# Autodesk Inventor assembly: GFRP_T2_02
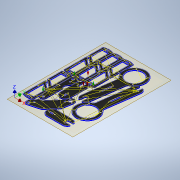
[picture p0: Inventor's stored thumbnail of the model, 180x180]
Saved by Autodesk Inventor 2022 (Build 260153000, 153)
## iProperties
Created: 2022-09-28
Part Number: GFRP_T2_02
Document SubType Name: Assembly
Designer: Masato
Author: Masato
## Documents named in this file (7)
- C:\Users\ヨコオリク\Documents\CITBrains\SUSTAINA-OP\Cam\GFRP_T2\OriginalMind_RD400\GFRP_T2_02.iam
- C:\Users\ヨコオリク\Documents\CITBrains\SUSTAINA-OP\Cam\DisposableBoard.ipt
- C:\Users\ヨコオリク\Documents\CITBrains\SUSTAINA-OP\LowerBody\Link\BackLink_frame.ipt
- C:\Users\ヨコオリク\Documents\CITBrains\SUSTAINA-OP\LowerBody\Link\FrontLink_frame.ipt
- C:\Users\ヨコオリク\Documents\CITBrains\SUSTAINA-OP\UpperBody\Arm\ForeArm_inside_frame.ipt
- C:\Users\ヨコオリク\Documents\CITBrains\SUSTAINA-OP\UpperBody\Arm\UpperArm_side_frame.ipt
- C:\Users\ヨコオリク\Documents\CITBrains\SUSTAINA-OP\UpperBody\Arm\ForeArm_outside_frame.ipt
## Components (15 placed, 6 different names)
1. DisposableBoard:1 — フラッシュ:1, フラッシュ:2, フラッシュ:3, フラッシュ:4, フラッシュ:9, 正接:11, 正接:12, フラッシュ:10, 正接:21, フラッシュ:13
2. BackLink_frame:4 — メイト:19, メイト:20, メイト:21, 正接:22
3. ForeArm_inside_frame:1 — メイト:11, 正接:25, フラッシュ:13
4. ForeArm_outside_frame:1 — メイト:10, 正接:11, 正接:12, 正接:13
5. UpperArm_side_frame:7 — メイト:16, 正接:18, メイト:19
6. UpperArm_side_frame:8 — メイト:17, 正接:18, フラッシュ:12, メイト:18, 正接:22, 正接:23
7. ForeArm_outside_frame:2 — 正接:7, 正接:9, 正接:10, 正接:13
8. FrontLink_frame:4 — メイト:13, 正接:21, 正接:24, 正接:25
9. ForeArm_inside_frame:2 — メイト:14, メイト:20, 正接:23, 正接:24
10. UpperArm_side_frame:4 — フラッシュ:7, 正接:6, フラッシュ:10, メイト:15
11. UpperArm_side_frame:1 — メイト:12, フラッシュ:7, フラッシュ:9, 正接:6, フラッシュ:12, メイト:18
12. UpperArm_side_frame:9
13. UpperArm_side_frame:10
14. UpperArm_side_frame:11 — 正接:7, 正接:10
15. UpperArm_side_frame:12 — 正接:9
## Component patterns: (3 elements, first: UpperArm_side_frame:4 + UpperArm_side_frame:1)
## Relationships (35: Tangent 13, Mate 12, Flush 10)
- フラッシュ:1 [Flush]: DisposableBoard:1
- フラッシュ:2 [Flush]: DisposableBoard:1
- フラッシュ:3 [Flush]: DisposableBoard:1
- フラッシュ:4 [Flush]: DisposableBoard:1
- メイト:10 [Mate]: ForeArm_outside_frame:1
- メイト:11 [Mate]: ForeArm_inside_frame:1
- メイト:12 [Mate]: UpperArm_side_frame:1
- フラッシュ:7 [Flush]: UpperArm_side_frame:4 ↔ UpperArm_side_frame:1
- [Flush]: UpperArm_side_frame:7 ↔ UpperArm_side_frame:8
- フラッシュ:9 [Flush] (2 mm): DisposableBoard:1 ↔ UpperArm_side_frame:1
- 正接:6 [Tangent] (2.1 mm): UpperArm_side_frame:4 ↔ UpperArm_side_frame:1
- 正接:7 [Tangent]: ForeArm_outside_frame:2 ↔ UpperArm_side_frame:11
- 正接:9 [Tangent] (2.1 mm): ForeArm_outside_frame:2 ↔ UpperArm_side_frame:12
- 正接:10 [Tangent] (2.1 mm): ForeArm_outside_frame:2 ↔ UpperArm_side_frame:11
- 正接:11 [Tangent] (2.1 mm): DisposableBoard:1 ↔ ForeArm_outside_frame:1
- 正接:12 [Tangent] (2.1 mm): DisposableBoard:1 ↔ ForeArm_outside_frame:1
- 正接:13 [Tangent] (2.1 mm): ForeArm_outside_frame:1 ↔ ForeArm_outside_frame:2
- メイト:13 [Mate]: FrontLink_frame:4
- メイト:14 [Mate]: ForeArm_inside_frame:2
- フラッシュ:10 [Flush] (-2.1 mm): DisposableBoard:1 ↔ UpperArm_side_frame:4
- メイト:15 [Mate]: UpperArm_side_frame:4
- メイト:16 [Mate]: UpperArm_side_frame:7
- メイト:17 [Mate]: UpperArm_side_frame:8
- メイト:18 [Mate] (2.1 mm): UpperArm_side_frame:8 ↔ UpperArm_side_frame:1
- 正接:18 [Tangent] (2.1 mm): UpperArm_side_frame:7 ↔ UpperArm_side_frame:8
- フラッシュ:12 [Flush]: UpperArm_side_frame:8 ↔ UpperArm_side_frame:1
- メイト:19 [Mate] (2.1 mm): BackLink_frame:4 ↔ UpperArm_side_frame:7
- 正接:21 [Tangent] (2 mm): DisposableBoard:1 ↔ FrontLink_frame:4
- メイト:20 [Mate] (2.1 mm): BackLink_frame:4 ↔ ForeArm_inside_frame:2
- メイト:21 [Mate]: BackLink_frame:4
- 正接:22 [Tangent]: BackLink_frame:4 ↔ UpperArm_side_frame:8
- 正接:23 [Tangent]: UpperArm_side_frame:8 ↔ ForeArm_inside_frame:2
- 正接:24 [Tangent] (2.1 mm): FrontLink_frame:4 ↔ ForeArm_inside_frame:2
- 正接:25 [Tangent] (2.1 mm): ForeArm_inside_frame:1 ↔ FrontLink_frame:4
- フラッシュ:13 [Flush] (-2 mm): DisposableBoard:1 ↔ ForeArm_inside_frame:1
## Named parameters: d52_d51 = 0 mm
